# Autodesk Inventor assembly: Ass_ServoGear
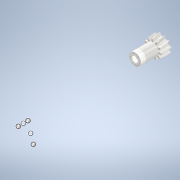
[picture p0: Inventor's stored thumbnail of the model, 180x180]
Saved by Autodesk Inventor 2022 (Build 260153000, 153)
## iProperties
Created: 2022-04-25
Part Number: Ass_ServoGear
Document SubType Name: Assembly
Designer: 32497
Author: 32497
## Documents named in this file (3)
- C:\Users\32497\OneDrive - Vrije Universiteit Brussel\Documents\3BA\Bachelorproef\OneDrive_2022-04-19\Shared Folder\CAD\V7\GearKlein.iam
- C:\Users\32497\OneDrive - Vrije Universiteit Brussel\Documents\3BA\Bachelorproef\OneDrive_2022-04-19\Shared Folder\CAD\V7\GearKleinPart1.ipt
- C:\Users\32497\OneDrive - Vrije Universiteit Brussel\Documents\3BA\Bachelorproef\OneDrive_2022-04-19\Shared Folder\CAD\V7\GearKleinPart2.ipt
## Components (2 placed, 2 different names)
1. GearKleinPart2:1 — Mate:1, Mate:2
2. Bevel Gear1:1 — Mate:1, Mate:2
## Relationships (2: Mate 2)
- Mate:1: GearKleinPart2:1 ↔ Bevel Gear1:1
- Mate:2: GearKleinPart2:1 ↔ Bevel Gear1:1
